# Autodesk Inventor assembly: suspension_one_side
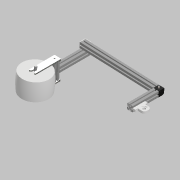
[picture p0: Inventor's stored thumbnail of the model, 180x180]
Saved by Autodesk Inventor 2021.2 (Build 252289000, 289)
## iProperties
Created: 2021-05-27
Part Number: suspension_one_side
Document SubType Name: Assembly
Designer: gisen
Author: gisen
## Documents named in this file (9)
- C:\Users\gisen\workspace\beetle_inventor_model\suspension\rocker_right.iam
- C:\Users\gisen\workspace\beetle_inventor_model\suspension\C-BGHKA6902ZZ-30\C-BGHKA6902ZZ-30.iam
- C:\Users\gisen\workspace\beetle_inventor_model\suspension\frame\AFS-3030-200.ipt
- C:\Users\gisen\workspace\beetle_inventor_model\suspension\wheel_with_mounts.iam
- C:\Users\gisen\workspace\beetle_inventor_model\suspension\frame\AFS-3030-174.ipt
- C:\Users\gisen\workspace\beetle_inventor_model\suspension\CAM\rocker_frame_mount_00.ipt
- C:\Users\gisen\workspace\beetle_inventor_model\suspension\CAM\rocker_frame_mount_01.ipt
- C:\Users\gisen\workspace\beetle_inventor_model\suspension\frame\AFS-3030-405.ipt
- C:\Users\gisen\workspace\beetle_inventor_model\suspension\frame\ABC-3030-6.ipt
## Components (8 placed, 8 different names)
1. C-BGHKA6902ZZ-30:1 [sub-assembly] — メイト:5, メイト:18, 角度:1, フラッシュ:15
2. AFS-3030-405:1 — メイト:5, フラッシュ:6, メイト:23, メイト:6, メイト:8, メイト:15, フラッシュ:9, メイト:17, フラッシュ:11, メイト:21, メイト:22
3. AFS-3030-174:1 — フラッシュ:6, メイト:23, メイト:6, メイト:18, 角度:1, フラッシュ:15, メイト:24
4. rocker_frame_mount_00:1 — メイト:8, メイト:16, メイト:17, フラッシュ:11
5. AFS-3030-200:1 — フラッシュ:16, メイト:25, メイト:14, メイト:15, フラッシュ:9, メイト:16, メイト:20, フラッシュ:14
6. wheel_with_mounts:1 [sub-assembly] — フラッシュ:16, メイト:25, メイト:14, フラッシュ:10
7. rocker_frame_mount_01:1 — メイト:20, メイト:21, フラッシュ:14
8. ABC-3030-6:1 — メイト:22, メイト:24
## Relationships (22: Mate 14, Flush 7, Angle 1)
- メイト:5 [Mate] (-15 mm): C-BGHKA6902ZZ-30:1 ↔ AFS-3030-405:1
- フラッシュ:6 [Flush]: AFS-3030-405:1 ↔ AFS-3030-174:1
- メイト:23 [Mate]: AFS-3030-405:1 ↔ AFS-3030-174:1
- メイト:6 [Mate]: AFS-3030-405:1 ↔ AFS-3030-174:1
- メイト:8 [Mate]: AFS-3030-405:1 ↔ rocker_frame_mount_00:1
- フラッシュ:16 [Flush]: AFS-3030-200:1 ↔ wheel_with_mounts:1
- メイト:25 [Mate] (33.5 mm): AFS-3030-200:1 ↔ wheel_with_mounts:1
- メイト:14 [Mate]: AFS-3030-200:1 ↔ wheel_with_mounts:1
- メイト:15 [Mate] (3 mm): AFS-3030-405:1 ↔ AFS-3030-200:1
- フラッシュ:9 [Flush]: AFS-3030-405:1 ↔ AFS-3030-200:1
- メイト:16 [Mate]: rocker_frame_mount_00:1 ↔ AFS-3030-200:1
- メイト:17 [Mate]: AFS-3030-405:1 ↔ rocker_frame_mount_00:1
- メイト:18 [Mate]: C-BGHKA6902ZZ-30:1 ↔ AFS-3030-174:1
- フラッシュ:10 [Flush]: wheel_with_mounts:1
- フラッシュ:11 [Flush]: AFS-3030-405:1 ↔ rocker_frame_mount_00:1
- メイト:20 [Mate]: AFS-3030-200:1 ↔ rocker_frame_mount_01:1
- メイト:21 [Mate]: AFS-3030-405:1 ↔ rocker_frame_mount_01:1
- フラッシュ:14 [Flush]: AFS-3030-200:1 ↔ rocker_frame_mount_01:1
- 角度:1 [Angle] (0 deg): C-BGHKA6902ZZ-30:1 ↔ AFS-3030-174:1
- フラッシュ:15 [Flush]: C-BGHKA6902ZZ-30:1 ↔ AFS-3030-174:1
- メイト:22 [Mate]: AFS-3030-405:1 ↔ ABC-3030-6:1
- メイト:24 [Mate]: AFS-3030-174:1 ↔ ABC-3030-6:1
